# Autodesk Inventor assembly: J002876
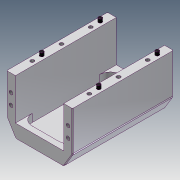
[picture p0: Inventor's stored thumbnail of the model, 180x180]
Saved by Autodesk Inventor 2015 SP1 (Build 190203100, 203)
## iProperties
Created: 2014-07-29
Vendor: HHMI: JFRC - ID&F
Document SubType Name: Assembly
Designer: arnoldj
Description: MPS SLING
Part Number: J002876
Project: P-194005
RuleStatus: InUse
AfterDocSave0: file://Part Number Cleaner
DESIGN DEPARTMENT: HHMI: JFRC - ID&F
LAB/DEPT: SVOBODA (LAB)
REQUESTING SCIENTIST: PERON, SIMON
SPECIAL FINISH: ANODIZE PER MIL-A-8625F, TYPE II, CLASS 2 (BLACK)
SURFACE ROUGHNESS: 63 Ra
ALTERED ITEM PART NUMBER: N/A
ALTERED ITEM VENDOR: N/A
ALTERED ITEM DESCRIPTION: N/A
Revision Number: 0
## Documents named in this file (3)
- C:\_WORKSPACE\DATA\PROJECTS\MOUSE POSITIONING SYSTEM\MCAD\STATIONARY SETUP\MPS Sling.iam
- C:\_WORKSPACE\DATA\PROJECTS\MOUSE POSITIONING SYSTEM\MCAD\STATIONARY SETUP\97395A441.ipt
- C:\_WORKSPACE\DATA\PROJECTS\MOUSE POSITIONING SYSTEM\MCAD\STATIONARY SETUP\MPS Sling.ipt
## Components (5 placed, 2 different names)
1. MPS Sling:1 — Mate:1, Mate:2, Mate:3, Flush:1, Mate:4, Flush:2, Mate:5, Flush:3
2. 97395A441:1 — Mate:1, Mate:2
3. 97395A441:2 — Mate:3, Flush:1
4. 97395A441:3 — Mate:4, Flush:2
5. 97395A441:4 — Mate:5, Flush:3
## Relationships (8: Mate 5, Flush 3)
- Mate:1: MPS Sling:1 ↔ 97395A441:1
- Mate:2 (3.175 mm): MPS Sling:1 ↔ 97395A441:1
- Mate:3: MPS Sling:1 ↔ 97395A441:2
- Flush:1 (-3.175 mm): MPS Sling:1 ↔ 97395A441:2
- Mate:4: MPS Sling:1 ↔ 97395A441:3
- Flush:2 (3.175 mm): MPS Sling:1 ↔ 97395A441:3
- Mate:5: MPS Sling:1 ↔ 97395A441:4
- Flush:3 (-3.175 mm): MPS Sling:1 ↔ 97395A441:4
